# Autodesk Inventor assembly: ETZ
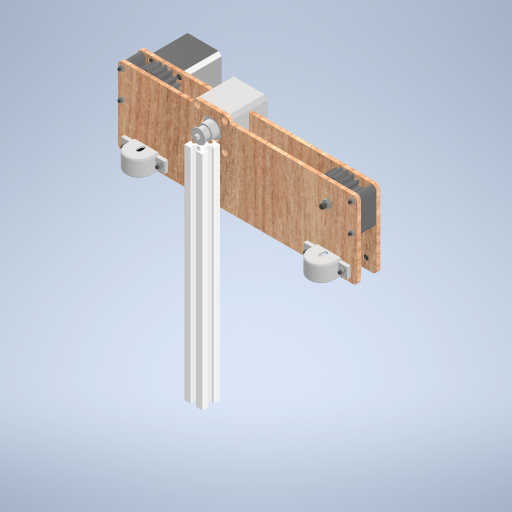
[picture p0: Inventor's stored thumbnail of the model, 512x512]
Saved by Autodesk Inventor 2024 (Build 280153000, 153)
## iProperties
Created: 2026-02-04
Part Number: ETZ
Document SubType Name: Assembly
Designer: SEMEN
Author: SEMEN
## Documents named in this file (3)
- C:\Users\SEMEN\Documents\ETZ2.0\ETZ.iam
- C:\Users\SEMEN\Documents\ETZ2.0\x_axis.iam
- C:\Users\SEMEN\Downloads\Assembly1.iam
## Components (2 placed, 2 different names)
1. x_axis:1 [sub-assembly] — Mate:1, Tangent:1
2. y_axis [sub-assembly] — Mate:1, Tangent:1
## Relationships (2: Mate 1, Tangent 1)
- Mate:1: x_axis:1 ↔ y_axis
- Tangent:1 (-2 mm): x_axis:1 ↔ y_axis
